# Autodesk Inventor assembly: full_fixed
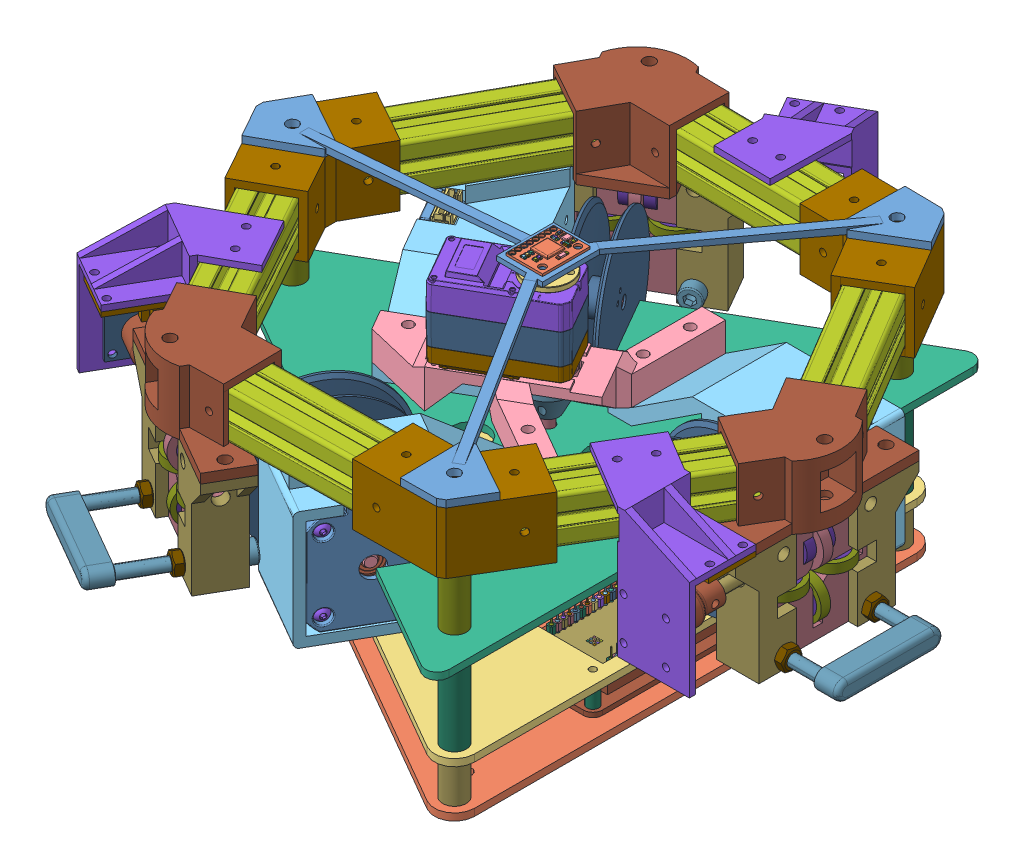
[picture p0: shaded view drawn from the shape stored in the file]
Saved by Autodesk Inventor 2024 (Build 280153000, 153)
## iProperties
Created: 2026-03-30
Part Number: full_fixed
Document SubType Name: Assembly
Designer: schar
Mass: 2163.44 g
Surface Area: 6584.11 cm^2
Volume: 1009.76 cm^3
Density: 2.14254 g/cm^3
Author: schar
## Documents named in this file (32)
- C:\Users\schar\Desktop\FloatingFace\models\full_fixed.iam
- C:\Users\schar\Desktop\FloatingFace\models\2020_nodes_conn.ipt
- C:\Users\schar\Desktop\FloatingFace\models\2020_extrusion.ipt
- C:\Users\schar\Desktop\FloatingFace\models\2020_top_guide_mnt.ipt
- C:\Users\schar\Desktop\FloatingFace\models\baseplate.ipt
- C:\Users\schar\Desktop\FloatingFace\models\spacer_2020_node.ipt
- C:\Users\schar\Desktop\FloatingFace\models\servo_holder.ipt
- C:\Users\schar\Desktop\FloatingFace\models\17HS4401S_Stepper_Motor\17HS4401S_Stepper_Motor.iam
- C:\Users\schar\Desktop\FloatingFace\models\nema_brackets_and_lineguides.ipt
- C:\Users\schar\Desktop\FloatingFace\models\spool.ipt
- C:\Users\schar\Desktop\FloatingFace\models\2020_guide_adaptor.ipt
- C:\Users\schar\Desktop\FloatingFace\models\guide.iam
- C:\Users\schar\Desktop\FloatingFace\models\spacer_etage.ipt
- C:\Users\schar\Desktop\FloatingFace\models\second_etage.ipt
- C:\Users\schar\Desktop\FloatingFace\models\esp_spacer_fixed.ipt
- C:\Users\schar\Desktop\FloatingFace\models\multifunctional_lvl.ipt
- C:\Users\schar\Downloads\ROBOTIC_DOG_-STEP\drivers_pcb_v1.1.ipt
- C:\Users\schar\Desktop\FloatingFace\models\esp_plate.ipt
- C:\Users\schar\Desktop\FloatingFace\models\servo_rod_connector.ipt
- C:\Users\schar\Desktop\FloatingFace\models\ST3215 Servo.iam
- C:\Users\schar\Desktop\FloatingFace\models\vertix_rod.ipt
- C:\Users\schar\Desktop\FloatingFace\models\esp32-s3-wroom-1-1.snapshot.2\ESP32-S3-WROOM-1\ESP32-S3-WROOM-1.iam
- C:\Users\schar\Desktop\FloatingFace\models\servo_board_spacer.ipt
- C:\Users\schar\Desktop\FloatingFace\models\multif_lvl_spacer.ipt
- C:\Users\schar\Desktop\FloatingFace\models\counter_sensors_assembly.iam
- C:\Users\schar\Desktop\FloatingFace\models\adafruit_TCA9548A_board.ipt
- C:\Users\schar\Desktop\FloatingFace\models\i2c_mplx_spacer.ipt
- C:\Users\schar\Desktop\FloatingFace\models\MPU6050 v2.ipt
- C:\Users\schar\Desktop\FloatingFace\models\mpu_unit_holder.ipt
- C:\Users\schar\Documents\Inventor\Content Center Files\R2024\en-US\DIN 912\DIN 912 - M5 x 0,8 x 40 x 22.ipt
- C:\Users\schar\Documents\Inventor\Content Center Files\R2024\en-US\DIN 934\DIN 934 - M5 x 0,8.ipt
- C:\Users\schar\Desktop\FloatingFace\models\stl\bumper.ipt
## Components (76 placed, 31 different names)
1. 2020_nodes_conn:1 — Mate:1, Mate:2, Mate:3, Mate:4, Mate:45, Mate:50, Mate:132, Flush:30
2. 2020_extrusion:1 — Mate:2, Mate:3, Mate:4, Mate:21, Mate:22, Mate:23, Flush:24, Mate:126, Flush:25
3. 2020_extrusion:2 — Mate:12, Mate:13, Mate:14, Mate:24, Mate:25, Mate:26
4. 2020_extrusion:3 — Mate:42, Mate:43, Mate:44
5. 2020_extrusion:4 — Mate:36, Mate:37, Mate:38, Mate:39, Mate:40, Mate:41, Mate:127, Flush:26
6. 2020_extrusion:5 — Mate:30, Mate:31, Mate:32, Mate:33, Mate:34, Mate:35, Flush:32
7. 2020_extrusion:6 — Mate:15, Mate:16, Mate:17, Mate:27, Mate:28, Mate:29, Mate:128, Flush:27
8. 2020_nodes_conn:2 — Mate:12, Mate:13, Mate:14, Mate:15, Mate:16, Mate:17, Mate:47, Mate:48
9. 2020_nodes_conn:3 — Mate:33, Mate:34, Mate:35, Mate:36, Mate:37, Mate:38, Mate:46, Mate:49
10. 2020_top_guide_mnt:1 — Mate:21, Mate:22, Mate:23, Mate:24, Mate:25, Mate:26, Flush:16, Mate:72, Flush:17
11. 2020_top_guide_mnt:2 — Mate:27, Mate:28, Mate:29, Mate:30, Mate:31, Mate:32, Mate:71, Flush:14, Flush:15
12. 2020_top_guide_mnt:3 — Mate:39, Mate:40, Mate:41, Mate:42, Mate:43, Mate:44, Mate:70, Flush:12, Flush:13
13. baseplate:1 — Mate:51, Mate:52, Mate:53, Mate:57, Mate:58, Mate:59, Mate:60, Mate:61, Mate:62, Mate:63, Mate:64, Mate:65, Mate:79, Mate:80, Mate:81, Mate:82, Mate:83, Mate:84, Mate:130, Angle:3
14. spacer_2020_node:1 — Mate:46, Mate:49, Mate:52, Mate:53
15. spacer_2020_node:2 — Mate:47, Mate:48
16. spacer_2020_node:3 — Mate:45, Mate:50, Mate:51
17. 17HS4401S_Stepper_Motor:1 [sub-assembly] — Mate:69, Mate:138, Mate:139, Angle:6
18. 17HS4401S_Stepper_Motor:2 [sub-assembly] — Mate:67, Mate:136, Mate:137, Angle:5
19. 17HS4401S_Stepper_Motor:3 [sub-assembly] — Mate:68, Mate:134, Mate:135, Angle:4
20. nema_brackets_and_lineguides:1 — Mate:60, Mate:61, Mate:62, Mate:66, Flush:7, Flush:8, Flush:9, Mate:136, Mate:137, Angle:5
21. nema_brackets_and_lineguides:2 — Mate:57, Mate:58, Mate:59, Flush:11, Mate:138, Mate:139, Angle:6
22. nema_brackets_and_lineguides:3 — Mate:63, Mate:64, Mate:65, Flush:10, Mate:134, Mate:135, Angle:4
23. servo_holder:1 — Mate:66, Flush:7, Flush:8, Mate:101, Mate:102, Angle:2
24. spool:1 — Mate:67, Flush:9
25. spool:2 — Mate:68, Flush:10
26. spool:3 — Mate:69, Flush:11
27. 2020_guide_adaptor:1 — Mate:70, Flush:12, Flush:13, Mate:73, Flush:18, Mate:74, Mate:143, Mate:144, Mate:146, Mate:148, Mate:150
28. 2020_guide_adaptor:2 — Mate:71, Flush:14, Flush:15, Mate:77, Mate:78, Flush:20, Mate:164, Mate:165, Mate:167, Mate:169
29. 2020_guide_adaptor:3 — Flush:16, Mate:72, Flush:17, Mate:75, Flush:19, Mate:76, Mate:153, Mate:154, Mate:155, Mate:156, Mate:157, Mate:158
30. guide:1 [sub-assembly] — Mate:75, Flush:19, Mate:76, Mate:140
31. guide:2 [sub-assembly] — Mate:77, Mate:78, Flush:20, Mate:141, Mate:162, Mate:163
32. guide:3 [sub-assembly] — Mate:73, Flush:18, Mate:74, Mate:142, Mate:145
33. spacer_etage:1 — Mate:80, Mate:84, Mate:87
34. spacer_etage:2 — Mate:79, Mate:83, Mate:85, Mate:86, Mate:131
35. spacer_etage:3 — Mate:81, Mate:82
36. second_etage:1 — Mate:85, Mate:86, Mate:87, Mate:88, Mate:89, Mate:90, Mate:91, Mate:92, Mate:93, Mate:94, Mate:95, Mate:96, Mate:97, Angle:1, Mate:109, Mate:110, Mate:111, Mate:112, Mate:113, Mate:114, Mate:115, Mate:116, Mate:117, Mate:118, Mate:119, Mate:120, Mate:121, Mate:122, Mate:129, Flush:28
37. esp_spacer_fixed:1 — Mate:88, Mate:95
38. esp_spacer_fixed:2 — Mate:89, Mate:93, Mate:99, Mate:100
39. esp_spacer_fixed:3 — Mate:91, Mate:92
40. esp_spacer_fixed:4 — Mate:90, Mate:94, Mate:98
41. multifunctional_lvl:1 — Mate:123, Mate:124, Mate:125
42. drivers_pcb_v1.1:1 — Mate:96, Mate:97, Angle:1
43. esp_plate:1 — Mate:98, Mate:99, Mate:100, Mate:108, Flush:21, Flush:22
44. servo_rod_connector:1 — Mate:103, Mate:104, Mate:105, Mate:106, Mate:107
45. ST3215 Servo:1 [sub-assembly] — Mate:101, Mate:102, Angle:2, Mate:103, Mate:104, Mate:105, Mate:133
46. vertix_rod:1 — Mate:106, Mate:107
47. ESP32-S3-WROOM-1:1 [sub-assembly] — Mate:108, Flush:21, Flush:22
48. servo_board_spacer:1 — Mate:109, Mate:115
49. servo_board_spacer:2 — Mate:110, Mate:114
50. servo_board_spacer:3 — Mate:112, Mate:113
51. servo_board_spacer:4 — Mate:111, Mate:116
52. multif_lvl_spacer:1 — Mate:117, Mate:122, Mate:125
53. multif_lvl_spacer:2 — Mate:118, Mate:121, Mate:124
54. multif_lvl_spacer:3 — Mate:119, Mate:120, Mate:123
55. counter_sensors_assembly:1 [sub-assembly] — Mate:126, Flush:25, Mate:140
56. counter_sensors_assembly:2 [sub-assembly] — Mate:127, Flush:26, Mate:142
57. counter_sensors_assembly:3 [sub-assembly] — Mate:128, Flush:27, Mate:141
58. adafruit_TCA9548A_board:1 — Mate:129, Mate:130, Mate:131
59. i2c_mplx_spacer:1 — Flush:28
60. MPU6050 v2:1 — Mate:132, Angle:3, Mate:133, Flush:29
61. mpu_unit_holder:1 — Flush:29, Flush:31
62. DIN 912 - replaced by DIN EN ISO 4762 M5 x 40:1 — Mate:143, Mate:144, Mate:149, Flush:33
63. DIN 912 - replaced by DIN EN ISO 4762 M5 x 40:2 — Mate:145, Mate:146, Mate:147
64. DIN 934 - replaced by DIN EN 24032/28673/28674 M5:1 — Mate:147, Mate:148
65. DIN 934 - replaced by DIN EN 24032/28673/28674 M5:2 — Mate:149, Mate:150
66. bumper:1 — Flush:33
67. DIN 912 - replaced by DIN EN ISO 4762 M5 x 40:3 — Mate:154, Mate:155, Mate:159, Mate:160
68. DIN 912 - replaced by DIN EN ISO 4762 M5 x 40:4 — Mate:153, Mate:156, Mate:161
69. DIN 934 - replaced by DIN EN 24032/28673/28674 M5:3 — Mate:157
70. DIN 934 - replaced by DIN EN 24032/28673/28674 M5:4 — Mate:158
71. bumper:2 — Mate:159, Mate:160, Mate:161
72. DIN 912 - replaced by DIN EN ISO 4762 M5 x 40:5 — Mate:163, Mate:164, Mate:166, Mate:170, Mate:172
73. DIN 912 - replaced by DIN EN ISO 4762 M5 x 40:6 — Mate:162, Mate:165, Mate:168, Mate:171
74. bumper:3 — Mate:170, Mate:171, Mate:172
75. DIN 934 - replaced by DIN EN 24032/28673/28674 M5:5 — Mate:166, Mate:167
76. DIN 934 - replaced by DIN EN 24032/28673/28674 M5:6 — Mate:168, Mate:169
## Relationships (191: Mate 159, Flush 26, Angle 6)
- Mate:1: 2020_nodes_conn:1
- Mate:2: 2020_nodes_conn:1 ↔ 2020_extrusion:1
- Mate:3: 2020_nodes_conn:1 ↔ 2020_extrusion:1
- Mate:4: 2020_nodes_conn:1 ↔ 2020_extrusion:1
- Mate:12: 2020_extrusion:2 ↔ 2020_nodes_conn:2
- Mate:13: 2020_extrusion:2 ↔ 2020_nodes_conn:2
- Mate:14: 2020_extrusion:2 ↔ 2020_nodes_conn:2
- Mate:15: 2020_extrusion:6 ↔ 2020_nodes_conn:2
- Mate:16: 2020_extrusion:6 ↔ 2020_nodes_conn:2
- Mate:17: 2020_extrusion:6 ↔ 2020_nodes_conn:2
- Mate:21: 2020_extrusion:1 ↔ 2020_top_guide_mnt:1
- Mate:22: 2020_extrusion:1 ↔ 2020_top_guide_mnt:1
- Mate:23: 2020_extrusion:1 ↔ 2020_top_guide_mnt:1
- Mate:24: 2020_extrusion:2 ↔ 2020_top_guide_mnt:1
- Mate:25: 2020_extrusion:2 ↔ 2020_top_guide_mnt:1
- Mate:26: 2020_extrusion:2 ↔ 2020_top_guide_mnt:1
- Mate:27: 2020_extrusion:6 ↔ 2020_top_guide_mnt:2
- Mate:28: 2020_extrusion:6 ↔ 2020_top_guide_mnt:2
- Mate:29: 2020_extrusion:6 ↔ 2020_top_guide_mnt:2
- Mate:30: 2020_extrusion:5 ↔ 2020_top_guide_mnt:2
- Mate:31: 2020_extrusion:5 ↔ 2020_top_guide_mnt:2
- Mate:32: 2020_extrusion:5 ↔ 2020_top_guide_mnt:2
- Mate:33: 2020_extrusion:5 ↔ 2020_nodes_conn:3
- Mate:34: 2020_extrusion:5 ↔ 2020_nodes_conn:3
- Mate:35: 2020_extrusion:5 ↔ 2020_nodes_conn:3
- Mate:36: 2020_extrusion:4 ↔ 2020_nodes_conn:3
- Mate:37: 2020_extrusion:4 ↔ 2020_nodes_conn:3
- Mate:38: 2020_extrusion:4 ↔ 2020_nodes_conn:3
- Mate:39: 2020_extrusion:4 ↔ 2020_top_guide_mnt:3
- Mate:40: 2020_extrusion:4 ↔ 2020_top_guide_mnt:3
- Mate:41: 2020_extrusion:4 ↔ 2020_top_guide_mnt:3
- Mate:42: 2020_extrusion:3 ↔ 2020_top_guide_mnt:3
- Mate:43: 2020_extrusion:3 ↔ 2020_top_guide_mnt:3
- Mate:44: 2020_extrusion:3 ↔ 2020_top_guide_mnt:3
- Mate:45: 2020_nodes_conn:1 ↔ spacer_2020_node:3
- Mate:46: 2020_nodes_conn:3 ↔ spacer_2020_node:1
- Mate:47: 2020_nodes_conn:2 ↔ spacer_2020_node:2
- Mate:48: 2020_nodes_conn:2 ↔ spacer_2020_node:2
- Mate:49: 2020_nodes_conn:3 ↔ spacer_2020_node:1
- Mate:50: 2020_nodes_conn:1 ↔ spacer_2020_node:3
- Mate:51: baseplate:1 ↔ spacer_2020_node:3
- Mate:52: baseplate:1 ↔ spacer_2020_node:1
- Mate:53: baseplate:1 ↔ spacer_2020_node:1
- Mate:57: baseplate:1 ↔ nema_brackets_and_lineguides:2
- Mate:58: baseplate:1 ↔ nema_brackets_and_lineguides:2
- Mate:59: baseplate:1 ↔ nema_brackets_and_lineguides:2
- Mate:60: baseplate:1 ↔ nema_brackets_and_lineguides:1
- Mate:61: baseplate:1 ↔ nema_brackets_and_lineguides:1
- Mate:62: baseplate:1 ↔ nema_brackets_and_lineguides:1
- Mate:63: baseplate:1 ↔ nema_brackets_and_lineguides:3
- Mate:64: baseplate:1 ↔ nema_brackets_and_lineguides:3
- Mate:65: baseplate:1 ↔ nema_brackets_and_lineguides:3
- Mate:66: nema_brackets_and_lineguides:1 ↔ servo_holder:1
- Flush:7: nema_brackets_and_lineguides:1 ↔ servo_holder:1
- Flush:8: nema_brackets_and_lineguides:1 ↔ servo_holder:1
- Mate:67: 17HS4401S_Stepper_Motor:2 ↔ spool:1
- Flush:9: nema_brackets_and_lineguides:1 ↔ spool:1
- Mate:68: 17HS4401S_Stepper_Motor:3 ↔ spool:2
- Flush:10: nema_brackets_and_lineguides:3 ↔ spool:2
- Mate:69: 17HS4401S_Stepper_Motor:1 ↔ spool:3
- Flush:11: nema_brackets_and_lineguides:2 ↔ spool:3
- Mate:70: 2020_top_guide_mnt:3 ↔ 2020_guide_adaptor:1
- Flush:12: 2020_top_guide_mnt:3 ↔ 2020_guide_adaptor:1
- Flush:13: 2020_top_guide_mnt:3 ↔ 2020_guide_adaptor:1
- Mate:71: 2020_top_guide_mnt:2 ↔ 2020_guide_adaptor:2
- Flush:14: 2020_top_guide_mnt:2 ↔ 2020_guide_adaptor:2
- Flush:15: 2020_top_guide_mnt:2 ↔ 2020_guide_adaptor:2
- Flush:16: 2020_top_guide_mnt:1 ↔ 2020_guide_adaptor:3
- Mate:72: 2020_top_guide_mnt:1 ↔ 2020_guide_adaptor:3
- Flush:17: 2020_top_guide_mnt:1 ↔ 2020_guide_adaptor:3
- Mate:73: 2020_guide_adaptor:1 ↔ guide:3
- Flush:18: 2020_guide_adaptor:1 ↔ guide:3
- Mate:74: 2020_guide_adaptor:1 ↔ guide:3
- Mate:75: 2020_guide_adaptor:3 ↔ guide:1
- Flush:19: 2020_guide_adaptor:3 ↔ guide:1
- Mate:76: 2020_guide_adaptor:3 ↔ guide:1
- Mate:77: 2020_guide_adaptor:2 ↔ guide:2
- Mate:78: 2020_guide_adaptor:2 ↔ guide:2
- Flush:20: 2020_guide_adaptor:2 ↔ guide:2
- Mate:79: baseplate:1 ↔ spacer_etage:2
- Mate:80: baseplate:1 ↔ spacer_etage:1
- Mate:81: baseplate:1 ↔ spacer_etage:3
- Mate:82: baseplate:1 ↔ spacer_etage:3
- Mate:83: baseplate:1 ↔ spacer_etage:2
- Mate:84: baseplate:1 ↔ spacer_etage:1
- Mate:85: spacer_etage:2 ↔ second_etage:1
- Mate:86: spacer_etage:2 ↔ second_etage:1
- Mate:87: spacer_etage:1 ↔ second_etage:1
- Mate:88: second_etage:1 ↔ esp_spacer_fixed:1
- Mate:89: second_etage:1 ↔ esp_spacer_fixed:2
- Mate:90: second_etage:1 ↔ esp_spacer_fixed:4
- Mate:91: second_etage:1 ↔ esp_spacer_fixed:3
- Mate:92: second_etage:1 ↔ esp_spacer_fixed:3
- Mate:93: second_etage:1 ↔ esp_spacer_fixed:2
- Mate:94: second_etage:1 ↔ esp_spacer_fixed:4
- Mate:95: second_etage:1 ↔ esp_spacer_fixed:1
- Mate:96: second_etage:1 ↔ drivers_pcb_v1.1:1
- Mate:97: second_etage:1 ↔ drivers_pcb_v1.1:1
- Angle:1 (0 deg): second_etage:1 ↔ drivers_pcb_v1.1:1
- Mate:98: esp_spacer_fixed:4 ↔ esp_plate:1
- Mate:99: esp_spacer_fixed:2 ↔ esp_plate:1
- Mate:100: esp_spacer_fixed:2 ↔ esp_plate:1
- Mate:101: servo_holder:1 ↔ ST3215 Servo:1
- Mate:102: servo_holder:1 ↔ ST3215 Servo:1
- Angle:2 (180 deg): servo_holder:1 ↔ ST3215 Servo:1
- Mate:103: servo_rod_connector:1 ↔ ST3215 Servo:1
- Mate:104: servo_rod_connector:1 ↔ ST3215 Servo:1
- Mate:105: servo_rod_connector:1 ↔ ST3215 Servo:1
- Mate:106: servo_rod_connector:1 ↔ vertix_rod:1
- Mate:107 (5 mm): servo_rod_connector:1 ↔ vertix_rod:1
- Mate:108: esp_plate:1 ↔ ESP32-S3-WROOM-1:1
- Flush:21: esp_plate:1 ↔ ESP32-S3-WROOM-1:1
- Flush:22: esp_plate:1 ↔ ESP32-S3-WROOM-1:1
- Mate:109: second_etage:1 ↔ servo_board_spacer:1
- Mate:110: second_etage:1 ↔ servo_board_spacer:2
- Mate:111: second_etage:1 ↔ servo_board_spacer:4
- Mate:112: second_etage:1 ↔ servo_board_spacer:3
- Mate:113: second_etage:1 ↔ servo_board_spacer:3
- Mate:114: second_etage:1 ↔ servo_board_spacer:2
- Mate:115: second_etage:1 ↔ servo_board_spacer:1
- Mate:116: second_etage:1 ↔ servo_board_spacer:4
- Mate:117: second_etage:1 ↔ multif_lvl_spacer:1
- Mate:118: second_etage:1 ↔ multif_lvl_spacer:2
- Mate:119: second_etage:1 ↔ multif_lvl_spacer:3
- Mate:120: second_etage:1 ↔ multif_lvl_spacer:3
- Mate:121: second_etage:1 ↔ multif_lvl_spacer:2
- Mate:122: second_etage:1 ↔ multif_lvl_spacer:1
- Mate:123: multifunctional_lvl:1 ↔ multif_lvl_spacer:3
- Mate:124: multifunctional_lvl:1 ↔ multif_lvl_spacer:2
- Mate:125: multifunctional_lvl:1 ↔ multif_lvl_spacer:1
- Flush:24: 2020_extrusion:1
- Mate:126: 2020_extrusion:1 ↔ counter_sensors_assembly:1
- Flush:25: 2020_extrusion:1 ↔ counter_sensors_assembly:1
- Mate:127: 2020_extrusion:4 ↔ counter_sensors_assembly:2
- Flush:26: 2020_extrusion:4 ↔ counter_sensors_assembly:2
- Mate:128: 2020_extrusion:6 ↔ counter_sensors_assembly:3
- Flush:27: 2020_extrusion:6 ↔ counter_sensors_assembly:3
- Mate:129 (3 mm): second_etage:1 ↔ adafruit_TCA9548A_board:1
- Mate:130: baseplate:1 ↔ adafruit_TCA9548A_board:1
- Mate:131 (22 mm): spacer_etage:2 ↔ adafruit_TCA9548A_board:1
- Flush:28: second_etage:1 ↔ i2c_mplx_spacer:1
- Mate:132 (10 mm): 2020_nodes_conn:1 ↔ MPU6050 v2:1
- Angle:3 (0 deg): baseplate:1 ↔ MPU6050 v2:1
- Mate:133: ST3215 Servo:1 ↔ MPU6050 v2:1
- Flush:29: MPU6050 v2:1 ↔ mpu_unit_holder:1
- Flush:30: 2020_nodes_conn:1
- Flush:31: mpu_unit_holder:1
- Mate:134: 17HS4401S_Stepper_Motor:3 ↔ nema_brackets_and_lineguides:3
- Mate:135: 17HS4401S_Stepper_Motor:3 ↔ nema_brackets_and_lineguides:3
- Angle:4 (-90 deg): 17HS4401S_Stepper_Motor:3 ↔ nema_brackets_and_lineguides:3
- Mate:136: 17HS4401S_Stepper_Motor:2 ↔ nema_brackets_and_lineguides:1
- Mate:137: 17HS4401S_Stepper_Motor:2 ↔ nema_brackets_and_lineguides:1
- Angle:5 (180 deg): 17HS4401S_Stepper_Motor:2 ↔ nema_brackets_and_lineguides:1
- Mate:138: 17HS4401S_Stepper_Motor:1 ↔ nema_brackets_and_lineguides:2
- Mate:139: 17HS4401S_Stepper_Motor:1 ↔ nema_brackets_and_lineguides:2
- Angle:6 (180 deg): 17HS4401S_Stepper_Motor:1 ↔ nema_brackets_and_lineguides:2
- Flush:32: 2020_extrusion:5
- Mate:140 (3 mm): guide:1 ↔ counter_sensors_assembly:1
- Mate:141 (3 mm): guide:2 ↔ counter_sensors_assembly:3
- Mate:142 (3 mm): guide:3 ↔ counter_sensors_assembly:2
- Mate:143: 2020_guide_adaptor:1 ↔ DIN 912 - replaced by DIN EN ISO 4762 M5 x 40:1
- Mate:144: 2020_guide_adaptor:1 ↔ DIN 912 - replaced by DIN EN ISO 4762 M5 x 40:1
- Mate:145: guide:3 ↔ DIN 912 - replaced by DIN EN ISO 4762 M5 x 40:2
- Mate:146: 2020_guide_adaptor:1 ↔ DIN 912 - replaced by DIN EN ISO 4762 M5 x 40:2
- Mate:147: DIN 912 - replaced by DIN EN ISO 4762 M5 x 40:2 ↔ DIN 934 - replaced by DIN EN 24032/28673/28674 M5:1
- Mate:148: 2020_guide_adaptor:1 ↔ DIN 934 - replaced by DIN EN 24032/28673/28674 M5:1
- Mate:149: DIN 912 - replaced by DIN EN ISO 4762 M5 x 40:1 ↔ DIN 934 - replaced by DIN EN 24032/28673/28674 M5:2
- Mate:150: 2020_guide_adaptor:1 ↔ DIN 934 - replaced by DIN EN 24032/28673/28674 M5:2
- Flush:33: DIN 912 - replaced by DIN EN ISO 4762 M5 x 40:1 ↔ bumper:1
- [Mate]: DIN 912 - replaced by DIN EN ISO 4762 M5 x 40:4 ↔ DIN 934 - replaced by DIN EN 24032/28673/28674 M5:3
- [Mate]: DIN 912 - replaced by DIN EN ISO 4762 M5 x 40:3 ↔ DIN 934 - replaced by DIN EN 24032/28673/28674 M5:4
- Mate:153: 2020_guide_adaptor:3 ↔ DIN 912 - replaced by DIN EN ISO 4762 M5 x 40:4
- Mate:154: 2020_guide_adaptor:3 ↔ DIN 912 - replaced by DIN EN ISO 4762 M5 x 40:3
- Mate:155: 2020_guide_adaptor:3 ↔ DIN 912 - replaced by DIN EN ISO 4762 M5 x 40:3
- Mate:156: 2020_guide_adaptor:3 ↔ DIN 912 - replaced by DIN EN ISO 4762 M5 x 40:4
- Mate:157: 2020_guide_adaptor:3 ↔ DIN 934 - replaced by DIN EN 24032/28673/28674 M5:3
- Mate:158: 2020_guide_adaptor:3 ↔ DIN 934 - replaced by DIN EN 24032/28673/28674 M5:4
- Mate:159: DIN 912 - replaced by DIN EN ISO 4762 M5 x 40:3 ↔ bumper:2
- Mate:160: DIN 912 - replaced by DIN EN ISO 4762 M5 x 40:3 ↔ bumper:2
- Mate:161: DIN 912 - replaced by DIN EN ISO 4762 M5 x 40:4 ↔ bumper:2
- Mate:162: guide:2 ↔ DIN 912 - replaced by DIN EN ISO 4762 M5 x 40:6
- Mate:163: guide:2 ↔ DIN 912 - replaced by DIN EN ISO 4762 M5 x 40:5
- Mate:164: 2020_guide_adaptor:2 ↔ DIN 912 - replaced by DIN EN ISO 4762 M5 x 40:5
- Mate:165: 2020_guide_adaptor:2 ↔ DIN 912 - replaced by DIN EN ISO 4762 M5 x 40:6
- Mate:166: DIN 912 - replaced by DIN EN ISO 4762 M5 x 40:5 ↔ DIN 934 - replaced by DIN EN 24032/28673/28674 M5:5
- Mate:167: 2020_guide_adaptor:2 ↔ DIN 934 - replaced by DIN EN 24032/28673/28674 M5:5
- Mate:168: DIN 912 - replaced by DIN EN ISO 4762 M5 x 40:6 ↔ DIN 934 - replaced by DIN EN 24032/28673/28674 M5:6
- Mate:169: 2020_guide_adaptor:2 ↔ DIN 934 - replaced by DIN EN 24032/28673/28674 M5:6
- Mate:170: DIN 912 - replaced by DIN EN ISO 4762 M5 x 40:5 ↔ bumper:3
- Mate:171: DIN 912 - replaced by DIN EN ISO 4762 M5 x 40:6 ↔ bumper:3
- Mate:172: DIN 912 - replaced by DIN EN ISO 4762 M5 x 40:5 ↔ bumper:3
## Named parameters: d214_d205 = 0 mm, d215_d206 = 0 mm, d216_d207 = 0 mm, d217_d209 = 0 mm, d218_d210 = 0 mm, d219_d211 = 0 mm
